# Autodesk Inventor assembly: Y Axis
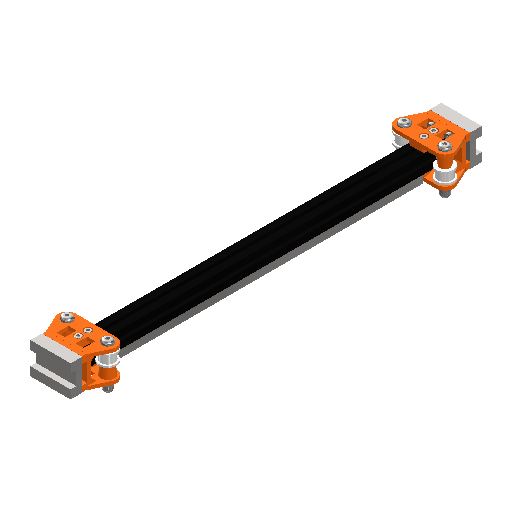
[picture p0: Inventor's stored thumbnail of the model, 512x512]
Saved by Autodesk Inventor 2023.2 (Build 272271000, 271)
## iProperties
Created: 2023-02-03
Part Number: Y Axis
Document SubType Name: Assembly
Designer: remop
Author: remop
## Documents named in this file (13)
- C:\Users\remop\OneDrive\Documents\Inventor\3D Printers\LuEVO\Mk5_FullKinematic\Y Axis.iam
- C:\Users\remop\OneDrive\Documents\Inventor\3D Printers\LuEVO\Mk5_FullKinematic\MGN12C.ipt
- C:\Users\remop\OneDrive\Documents\Inventor\3D Printers\LuEVO\Mk5_FullKinematic\Y Axis Gantry Spacer.ipt
- C:\Users\remop\OneDrive\Documents\Inventor\3D Printers\LuEVO\Mk5_FullKinematic\Y Axis Gantry Baseblock (CNC).ipt
- C:\Users\remop\OneDrive\Documents\Inventor\3D Printers\LuEVO\Mk5_FullKinematic\Makerbeam\Beam_320mm.ipt
- C:\Users\remop\OneDrive\Documents\Inventor\3D Printers\LuEVO\Mk5_FullKinematic\6mm smooth idler.ipt
- C:\Users\remop\OneDrive\Documents\Inventor\Content Center Files\R2023\en-US\AS 1420\AS 1420 - 1973 - M3 x 10.ipt
- C:\Users\remop\OneDrive\Documents\Inventor\3D Printers\LuEVO\Mk5_FullKinematic\MGNR12_275mm.ipt
- C:\Users\remop\OneDrive\Documents\Inventor\Content Center Files\R2023\en-US\AS 1237 (2.1)\AS 1237 - 5.ipt
- C:\Users\remop\OneDrive\Documents\Inventor\Content Center Files\R2023\en-US\AS 1420\AS 1420 - 1973 - M3 x 8.ipt
- C:\Users\remop\OneDrive\Documents\Inventor\Content Center Files\R2023\en-US\BS 4168(6)\BS 4168 - M5 x 30(6).ipt
- C:\Users\remop\OneDrive\Documents\Inventor\Content Center Files\R2023\en-US\DIN 1587\DIN 1587 - M5 x 0.8.ipt
- C:\Users\remop\OneDrive\Documents\Inventor\3D Printers\LuEVO\Mk5_FullKinematic\Idler Spacer.ipt
## Components (36 placed, 12 different names)
1. MGN12C:1 — Mate:1, Flush:1, Flush:2, Rigid:4
2. MGN12C:2 — Mate:1, Flush:1, Flush:2, Flush:3, Rigid:1
3. Y Axis Gantry Spacer:1 — Flush:3, Rigid:1, Rigid:2
4. Y Axis Gantry Baseblock (CNC):1 — Rigid:2, Mate:5, Insert:7, Insert:8, Insert:11, Insert:12, Insert:17, Insert:18, Insert:19, Insert:20, Rigid:11, Rigid:12
5. Y Axis Gantry Spacer:2 — Rigid:4, Rotational:1, Rotational:2
6. Y Axis Gantry Baseblock (CNC):2 — Mate:2, Insert:3, Insert:4, Insert:5, Insert:6, Mate:3, Flush:4, Insert:9, Insert:10, Insert:13, Insert:14, Rotational:1, Rotational:2, Insert:15, Insert:16, Insert:21, Insert:22, Rigid:9, Rigid:10
7. Beam_320mm:1 — Mate:2, Mate:3, Flush:4, Mate:4, Flush:5
8. AS 1420 - Metric M3 x 10:1 — Insert:3
9. AS 1420 - Metric M3 x 10:2 — Insert:4
10. AS 1420 - Metric M3 x 10:3 — Insert:5
11. AS 1420 - Metric M3 x 10:4 — Insert:6
12. MGNR12_275mm:1 — Mate:4, Mate:5, Flush:5
13. AS 1237 (2.1) 5:1 — Insert:7, Rigid:7
14. AS 1237 (2.1) 5:2 — Insert:8, Rigid:8
15. AS 1237 (2.1) 5:3 — Insert:9, Rigid:5
16. AS 1237 (2.1) 5:4 — Insert:10, Rigid:6
17. 6mm smooth idler:1 — Rigid:6
18. 6mm smooth idler:2 — Rigid:5
19. 6mm smooth idler:3 — Rigid:7
20. 6mm smooth idler:4 — Rigid:8
21. AS 1420 - Metric M3 x 8:1 — Insert:11
22. AS 1420 - Metric M3 x 8:2 — Insert:12
23. AS 1420 - Metric M3 x 8:3 — Insert:13
24. AS 1420 - Metric M3 x 8:4 — Insert:14
25. BS 4168 : Part 6 Hexagon socket countersunk and button head screws - Metric series - Metric M5 x 30:1 — Insert:15
26. BS 4168 : Part 6 Hexagon socket countersunk and button head screws - Metric series - Metric M5 x 30:2 — Insert:16
27. BS 4168 : Part 6 Hexagon socket countersunk and button head screws - Metric series - Metric M5 x 30:3 — Insert:17
28. BS 4168 : Part 6 Hexagon socket countersunk and button head screws - Metric series - Metric M5 x 30:4 — Insert:18
29. DIN 1587 M5:1 — Insert:19
30. DIN 1587 M5:2 — Insert:20
31. DIN 1587 M5:3 — Insert:21
32. DIN 1587 M5:4 — Insert:22
33. Idler Spacer:1 — Rigid:9
34. Idler Spacer:2 — Rigid:10
35. Idler Spacer:3 — Rigid:11
36. Idler Spacer:4 — Rigid:12
## Relationships (43: Insert 20, WeldJoint 11, Mate 5, Flush 5, RevoluteJoint 2)
- Mate:1 (334 mm): MGN12C:1 ↔ MGN12C:2
- Flush:1: MGN12C:1 ↔ MGN12C:2
- Flush:2: MGN12C:1 ↔ MGN12C:2
- Flush:3: MGN12C:2 ↔ Y Axis Gantry Spacer:1
- Rigid:1 [WeldJoint]: MGN12C:2 ↔ Y Axis Gantry Spacer:1
- Rigid:2 [WeldJoint]: Y Axis Gantry Spacer:1 ↔ Y Axis Gantry Baseblock (CNC):1
- Rigid:4 [WeldJoint]: MGN12C:1 ↔ Y Axis Gantry Spacer:2
- Mate:2: Y Axis Gantry Baseblock (CNC):2 ↔ Beam_320mm:1
- Insert:3: Y Axis Gantry Baseblock (CNC):2 ↔ AS 1420 - Metric M3 x 10:1
- Insert:4: Y Axis Gantry Baseblock (CNC):2 ↔ AS 1420 - Metric M3 x 10:2
- Insert:5: Y Axis Gantry Baseblock (CNC):2 ↔ AS 1420 - Metric M3 x 10:3
- Insert:6: Y Axis Gantry Baseblock (CNC):2 ↔ AS 1420 - Metric M3 x 10:4
- Mate:3: Y Axis Gantry Baseblock (CNC):2 ↔ Beam_320mm:1
- Flush:4 (10 mm): Y Axis Gantry Baseblock (CNC):2 ↔ Beam_320mm:1
- Mate:4: Beam_320mm:1 ↔ MGNR12_275mm:1
- Mate:5 (0.2 mm): Y Axis Gantry Baseblock (CNC):1 ↔ MGNR12_275mm:1
- Flush:5 (1.5 mm): Beam_320mm:1 ↔ MGNR12_275mm:1
- Insert:7: Y Axis Gantry Baseblock (CNC):1 ↔ AS 1237 (2.1) 5:1
- Insert:8: Y Axis Gantry Baseblock (CNC):1 ↔ AS 1237 (2.1) 5:2
- Insert:9: Y Axis Gantry Baseblock (CNC):2 ↔ AS 1237 (2.1) 5:3
- Insert:10: Y Axis Gantry Baseblock (CNC):2 ↔ AS 1237 (2.1) 5:4
- Rigid:5 [WeldJoint]: AS 1237 (2.1) 5:3 ↔ 6mm smooth idler:2
- Rigid:6 [WeldJoint]: AS 1237 (2.1) 5:4 ↔ 6mm smooth idler:1
- Rigid:7 [WeldJoint]: AS 1237 (2.1) 5:1 ↔ 6mm smooth idler:3
- Rigid:8 [WeldJoint]: AS 1237 (2.1) 5:2 ↔ 6mm smooth idler:4
- Insert:11: Y Axis Gantry Baseblock (CNC):1 ↔ AS 1420 - Metric M3 x 8:1
- Insert:12: Y Axis Gantry Baseblock (CNC):1 ↔ AS 1420 - Metric M3 x 8:2
- Insert:13: Y Axis Gantry Baseblock (CNC):2 ↔ AS 1420 - Metric M3 x 8:3
- Insert:14: Y Axis Gantry Baseblock (CNC):2 ↔ AS 1420 - Metric M3 x 8:4
- Rotational:1 [RevoluteJoint]: Y Axis Gantry Spacer:2 ↔ Y Axis Gantry Baseblock (CNC):2
- Rotational:2 [RevoluteJoint]: Y Axis Gantry Spacer:2 ↔ Y Axis Gantry Baseblock (CNC):2
- Insert:15: Y Axis Gantry Baseblock (CNC):2 ↔ BS 4168 : Part 6 Hexagon socket countersunk and button head screws - Metric series - Metric M5 x 30:1
- Insert:16: Y Axis Gantry Baseblock (CNC):2 ↔ BS 4168 : Part 6 Hexagon socket countersunk and button head screws - Metric series - Metric M5 x 30:2
- Insert:17: Y Axis Gantry Baseblock (CNC):1 ↔ BS 4168 : Part 6 Hexagon socket countersunk and button head screws - Metric series - Metric M5 x 30:3
- Insert:18: Y Axis Gantry Baseblock (CNC):1 ↔ BS 4168 : Part 6 Hexagon socket countersunk and button head screws - Metric series - Metric M5 x 30:4
- Insert:19: Y Axis Gantry Baseblock (CNC):1 ↔ DIN 1587 M5:1
- Insert:20: Y Axis Gantry Baseblock (CNC):1 ↔ DIN 1587 M5:2
- Insert:21: Y Axis Gantry Baseblock (CNC):2 ↔ DIN 1587 M5:3
- Insert:22: Y Axis Gantry Baseblock (CNC):2 ↔ DIN 1587 M5:4
- Rigid:9 [WeldJoint]: Y Axis Gantry Baseblock (CNC):2 ↔ Idler Spacer:1
- Rigid:10 [WeldJoint]: Y Axis Gantry Baseblock (CNC):2 ↔ Idler Spacer:2
- Rigid:11 [WeldJoint]: Y Axis Gantry Baseblock (CNC):1 ↔ Idler Spacer:3
- Rigid:12 [WeldJoint]: Y Axis Gantry Baseblock (CNC):1 ↔ Idler Spacer:4
